# Autodesk Inventor assembly: манипулятогр
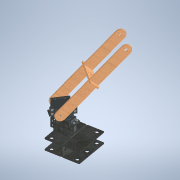
[picture p0: Inventor's stored thumbnail of the model, 180x180]
Saved by Autodesk Inventor 2020.1 (Build 241239000, 239)
## iProperties
Created: 2021-08-17
Part Number: манипулятогр
Document SubType Name: Assembly
Designer: Ni3na
Author: Ni3na
## Documents named in this file (4)
- D:\GitHub\avatar-kvantoriada\3D\манипулятогр .iam
- D:\GitHub\avatar-kvantoriada\3D\сборка серва.iam
- D:\GitHub\avatar-kvantoriada\3D\основа.ipt
- D:\GitHub\avatar-kvantoriada\3D\Сборка1.iam
## Components (5 placed, 3 different names)
1. сборка серва:1 [sub-assembly] — Жесткий:1, Жесткий:3
2. сборка серва:2 [sub-assembly] — Жесткий:1, Жесткий:5
3. основа:1 — Жесткий:3, Жесткий:4
4. основа:2 — Жесткий:4
5. Сборка1:1 [sub-assembly] — Жесткий:5
## Relationships (4: WeldJoint 4)
- Жесткий:1 [WeldJoint]: сборка серва:1 ↔ сборка серва:2
- Жесткий:3 [WeldJoint]: сборка серва:1 ↔ основа:1
- Жесткий:4 [WeldJoint]: основа:1 ↔ основа:2
- Жесткий:5 [WeldJoint]: сборка серва:2 ↔ Сборка1:1
